# Autodesk Inventor assembly: Assembly_layered_chip
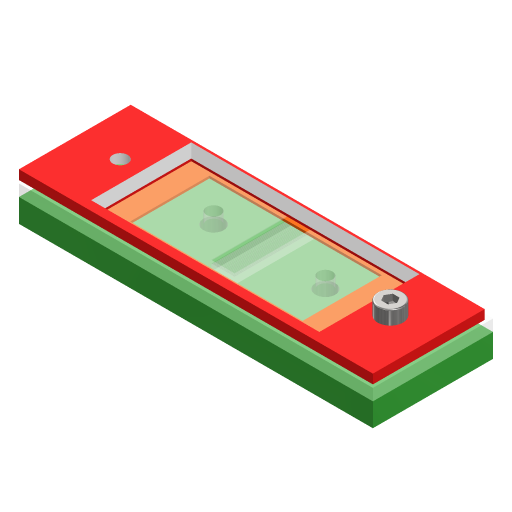
[picture p0: Inventor's stored thumbnail of the model, 512x512]
Saved by Autodesk Inventor 2024.1 (Build 281209000, 209)
## iProperties
Created: 2024-08-02
Part Number: Assembly_layered_chip
Document SubType Name: Assembly
Designer: diederichbenedict
Author: diederichbenedict
## Documents named in this file (7)
- C:\Users\diederichbenedict\Dropbox\Dokumente\Promotion\PROJECTS\TIRFImager\INVENTOR\Assembly_layered_chip.iam
- C:\Users\diederichbenedict\Dropbox\Dokumente\Promotion\PROJECTS\TIRFImager\INVENTOR\00_chipnano_waveguide_slidsize_modified.ipt
- C:\Users\diederichbenedict\Dropbox\Dokumente\Promotion\PROJECTS\TIRFImager\INVENTOR\00_Gasket.ipt
- C:\Users\diederichbenedict\Dropbox\Dokumente\Promotion\PROJECTS\TIRFImager\INVENTOR\00_coverglass_frame.ipt
- C:\Users\diederichbenedict\Dropbox\Dokumente\Promotion\PROJECTS\TIRFImager\INVENTOR\00_coverglass_50x22.ipt
- C:\Users\diederichbenedict\Dropbox\Dokumente\Promotion\PROJECTS\TIRFImager\INVENTOR\00_Sandwich_base.ipt
- C:\Users\diederichbenedict\Documents\Inventor\Content Center Files\R2024\de-DE\DIN 912\DIN 912 - M3 x 0.5 x 6 x 4.75.ipt
## Components (6 placed, 6 different names)
1. 00_chipnano_waveguide_slidsize_modified:1 — Fluchtend:1, Fluchtend:2, Fluchtend:3, Fluchtend:4, Fluchtend:7, Fluchtend:8
2. 00_Gasket:1 — Fluchtend:1, Fluchtend:2
3. 00_coverglass_50x22:1 — Fluchtend:3, Fluchtend:4, Fluchtend:5, Fluchtend:6
4. 00_coverglass_frame:1 — Fluchtend:5, Fluchtend:6, Einfügen:1
5. 00_Sandwich_base:1 — Fluchtend:7, Fluchtend:8
6. DIN 912 - ersetzt durch DIN EN ISO 4762 M3 x 6:1 — Einfügen:1
## Relationships (9: Flush 8, Insert 1)
- Fluchtend:1 [Flush]: 00_chipnano_waveguide_slidsize_modified:1 ↔ 00_Gasket:1
- Fluchtend:2 [Flush]: 00_chipnano_waveguide_slidsize_modified:1 ↔ 00_Gasket:1
- Fluchtend:3 [Flush]: 00_chipnano_waveguide_slidsize_modified:1 ↔ 00_coverglass_50x22:1
- Fluchtend:4 [Flush] (0.5 mm): 00_chipnano_waveguide_slidsize_modified:1 ↔ 00_coverglass_50x22:1
- Fluchtend:5 [Flush]: 00_coverglass_50x22:1 ↔ 00_coverglass_frame:1
- Fluchtend:6 [Flush]: 00_coverglass_50x22:1 ↔ 00_coverglass_frame:1
- Fluchtend:7 [Flush]: 00_chipnano_waveguide_slidsize_modified:1 ↔ 00_Sandwich_base:1
- Fluchtend:8 [Flush]: 00_chipnano_waveguide_slidsize_modified:1 ↔ 00_Sandwich_base:1
- Einfügen:1 [Insert]: 00_coverglass_frame:1 ↔ DIN 912 - ersetzt durch DIN EN ISO 4762 M3 x 6:1
